# Autodesk Inventor assembly: robot
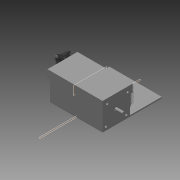
[picture p0: Inventor's stored thumbnail of the model, 180x180]
Saved by Autodesk Inventor 2015 (Build 190159000, 159)
## iProperties
Created: 2015-02-18
Part Number: robot
Document SubType Name: Assembly
Designer: jorge
Author: jorge
## Documents named in this file (7)
- \\psf\Home\Documents\proyectos\cybertech\sumo2015\diseno\robot.iam
- \\psf\Home\Documents\proyectos\cybertech\sumo2015\diseno\motor.ipt
- \\psf\Home\Documents\proyectos\cybertech\sumo2015\diseno\base.ipt
- \\psf\Home\Documents\proyectos\cybertech\sumo2015\diseno\king-max-1000-mah-lipo-battery-pack\Imported Components\bateria KingMax1000\bateria KingMax1000.ipt
- \\psf\Home\Documents\proyectos\cybertech\sumo2015\diseno\arduino-nano-microcontroller-1\Imported Components\Arduino Mini ASSY\Arduino Mini ASSY.iam
- \\psf\Home\Documents\proyectos\cybertech\sumo2015\diseno\mg90s-servo-1\Imported Components\MG90s_servo\MG90s_servo.ipt
- \\psf\Home\Documents\proyectos\cybertech\sumo2015\diseno\tapa.ipt
## Components (7 placed, 6 different names)
1. motor:1
2. motor:2
3. base:1
4. bateria KingMax1000:1
5. Arduino Mini ASSY:1 [sub-assembly]
6. MG90s_servo:1 — Rígido:1
7. tapa:1 — Rígido:1
## Relationships (1: WeldJoint 1)
- Rígido:1 [WeldJoint]: MG90s_servo:1 ↔ tapa:1
